# Autodesk Inventor assembly: COXA_PITCH_DRIVER_PULLEY
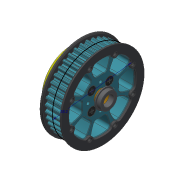
[picture p0: Inventor's stored thumbnail of the model, 180x180]
Saved by Autodesk Inventor 2019.4 (Build 234330000, 330)
## iProperties
Created: 2019-11-13
Part Number: COXA_PITCH_DRIVER_PULLEY
Material: 一般
Document SubType Name: Assembly
Designer: y6tada
Author: y6tada
## Documents named in this file (9)
- C:\Workspace\Yuni9\Inventor\Asm\UPPER_LEG\COXA_PITCH_DRIVER_PULLEY.iam
- C:\Workspace\Yuni9\Inventor\Ref\DDA Series\NMB_A2015\A-2015.iam
- C:\Workspace\Yuni9\Inventor\Asm\UPPER_LEG\COXA_PITCH_BEARING_BASE.ipt
- C:\Workspace\Yuni9\Inventor\Asm\UPPER_LEG\UPPER_TIMING_PULLEY_P40.ipt
- C:\Workspace\Yuni9\Inventor\Asm\UPPER_LEG\UPPER_TIMING_PULLEY_COVER_OUTER.ipt
- C:\Workspace\Yuni9\Inventor\Asm\UPPER_LEG\CB-501.5PC.ipt
- C:\Users\y6tada\Documents\Inventor\Content Center Files\R2019\ja-JP\ISO 7046-1 H(1)\ISO 7046-1 - M2 x 14 - 4.8 - H - ISO.ipt
- C:\Workspace\Yuni9\Inventor\Ref\NSK Bearing\NSK_RB_MF85ZZ\MF85ZZ.iam
- C:\Workspace\Yuni9\Inventor\Asm\UPPER_LEG\UPPER_TIMING_PULLEY_COVER_INNER.ipt
## Components (11 placed, 8 different names)
1. UPPER_TIMING_PULLEY_P40:1 — メイト:17, メイト:18, メイト:19, メイト:20
2. A-2015:1 [sub-assembly]
3. COXA_PITCH_BEARING_BASE:1 — メイト:16
4. UPPER_TIMING_PULLEY_COVER_OUTER:1
5. CB-501.5PC:1
6. ISO 7046-1 H M2 x 14 - 4.8 - H:1
7. ISO 7046-1 H M2 x 14 - 4.8 - H:2
8. ISO 7046-1 H M2 x 14 - 4.8 - H:3
9. ISO 7046-1 H M2 x 14 - 4.8 - H:4
10. MF85ZZ:1 [sub-assembly]
11. UPPER_TIMING_PULLEY_COVER_INNER:1 — メイト:19, メイト:20
## Relationships (21: Mate 20, Flush 1)
- [Mate]: A-2015:1 ↔ COXA_PITCH_BEARING_BASE:1
- [Mate]: UPPER_TIMING_PULLEY_P40:1 ↔ COXA_PITCH_BEARING_BASE:1
- [Mate]: UPPER_TIMING_PULLEY_P40:1 ↔ COXA_PITCH_BEARING_BASE:1
- [Mate]: UPPER_TIMING_PULLEY_P40:1 ↔ COXA_PITCH_BEARING_BASE:1
- [Flush]: UPPER_TIMING_PULLEY_P40:1 ↔ UPPER_TIMING_PULLEY_COVER_OUTER:1
- [Mate]: UPPER_TIMING_PULLEY_P40:1 ↔ UPPER_TIMING_PULLEY_COVER_OUTER:1
- [Mate]: UPPER_TIMING_PULLEY_P40:1 ↔ UPPER_TIMING_PULLEY_COVER_OUTER:1
- [Mate]: UPPER_TIMING_PULLEY_P40:1 ↔ UPPER_TIMING_PULLEY_COVER_OUTER:1
- [Mate]: UPPER_TIMING_PULLEY_P40:1 ↔ CB-501.5PC:1
- [Mate]: UPPER_TIMING_PULLEY_P40:1 ↔ CB-501.5PC:1
- [Mate]: UPPER_TIMING_PULLEY_P40:1 ↔ ISO 7046-1 H M2 x 14 - 4.8 - H:1
- [Mate]: UPPER_TIMING_PULLEY_P40:1 ↔ ISO 7046-1 H M2 x 14 - 4.8 - H:2
- [Mate]: UPPER_TIMING_PULLEY_P40:1 ↔ ISO 7046-1 H M2 x 14 - 4.8 - H:3
- [Mate]: UPPER_TIMING_PULLEY_P40:1 ↔ ISO 7046-1 H M2 x 14 - 4.8 - H:4
- [Mate]: CB-501.5PC:1 ↔ MF85ZZ:1
- [Mate]: CB-501.5PC:1 ↔ MF85ZZ:1
- メイト:16 [Mate]: COXA_PITCH_BEARING_BASE:1
- メイト:17 [Mate]: UPPER_TIMING_PULLEY_P40:1
- メイト:18 [Mate]: UPPER_TIMING_PULLEY_P40:1
- メイト:19 [Mate]: UPPER_TIMING_PULLEY_P40:1 ↔ UPPER_TIMING_PULLEY_COVER_INNER:1
- メイト:20 [Mate]: UPPER_TIMING_PULLEY_P40:1 ↔ UPPER_TIMING_PULLEY_COVER_INNER:1
## Named parameters: d0_d9 = 0 mm, d1_d10 = 0 mm, d2_d11 = 0 mm, d3_d12 = 0 mm, d4_d14 = 0 mm, d5_d15 = 0 mm
